# Autodesk Inventor assembly: korp
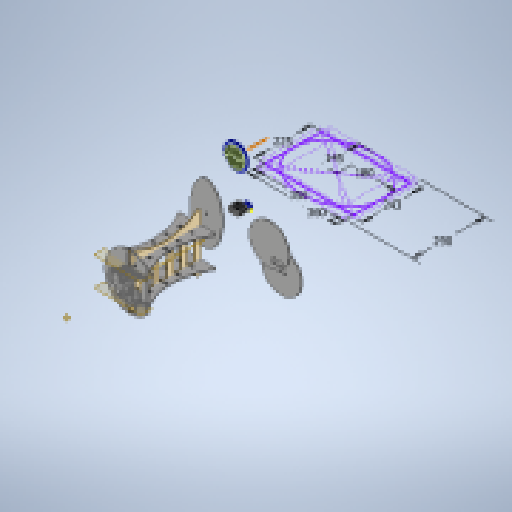
[picture p0: Inventor's stored thumbnail of the model, 512x512]
Saved by Autodesk Inventor 2023.1 (Build 271208000, 208)
## iProperties
Created: 2023-03-13
Part Number: korp
Document SubType Name: Assembly
Designer: User
Author: User
## Documents named in this file (18)
- C:\Users\DELL\reposGitHub\Cheburashka\Cheburashka_construction\korpus\korp.iam
- C:\Users\DELL\reposGitHub\Cheburashka\Cheburashka_construction\korpus\нижний эллипс тела.ipt
- C:\Users\DELL\reposGitHub\Cheburashka\Cheburashka_construction\korpus\грань тела.ipt
- C:\Users\DELL\reposGitHub\Cheburashka\Cheburashka_construction\korpus\верхний эллипс туловища.ipt
- C:\Users\DELL\reposGitHub\Cheburashka\Cheburashka_construction\korpus\нижний эллипс головы.ipt
- C:\Users\DELL\reposGitHub\Cheburashka\Cheburashka_construction\korpus\Servo.ipt
- C:\Users\DELL\reposGitHub\Cheburashka\Cheburashka_construction\korpus\Pitsco Education-739028.ipt
- C:\Users\DELL\reposGitHub\Cheburashka\Cheburashka_construction\korpus\Pitsco Education-739085.ipt
- C:\Users\DELL\reposGitHub\Cheburashka\Cheburashka_construction\korpus\трубка.ipt
- C:\Users\DELL\reposGitHub\Cheburashka\Cheburashka_construction\korpus\Prostavka.ipt
- C:\Users\DELL\reposGitHub\Cheburashka\Cheburashka_construction\korpus\лицо1.ipt
- C:\Users\DELL\reposGitHub\Cheburashka\Cheburashka_construction\korpus\att_pin.ipt
- C:\Users\DELL\reposGitHub\Cheburashka\Cheburashka_construction\platform\print\Деталь1.ipt
- C:\Users\DELL\reposGitHub\Cheburashka\Cheburashka_construction\platform\KRAVT_holder_2 (1).ipt
- C:\Users\DELL\reposGitHub\Cheburashka\Cheburashka_construction\korpus\ребро.ipt
- C:\Users\DELL\reposGitHub\Cheburashka\Cheburashka_construction\korpus\ребро_MIR.ipt
- C:\Users\DELL\reposGitHub\Cheburashka\Cheburashka_construction\korpus\креп.ipt
- C:\Users\DELL\reposGitHub\Cheburashka\Cheburashka_construction\korpus\креп_MIR.ipt
## Components (32 placed, 17 different names)
1. нижний эллипс тела:1 — Совмещение:100, Симметрия:1
2. верхний эллипс туловища:1
3. грань тела:1 — Совмещение:101, Заподлицо:19
4. нижний эллипс головы:1 — Совмещение:73
5. Pitsco Education-739028:1 — Совмещение:99
6. Pitsco Education-739085:1 — Совмещение:68, Совмещение:75, Совмещение:80
7. трубка:1 — Совмещение:68, Совмещение:74, Совмещение:81
8. Servo:4 — Совмещение:97, Совмещение:98
9. Prostavka:1 — Совмещение:73, Совмещение:74, Совмещение:75
10. Prostavka:2 — Совмещение:80, Совмещение:81, Заподлицо:16
11. лицо1:1 — Заподлицо:16, Заподлицо:17
12. att_pin:1 — Совмещение:97, Совмещение:98, Совмещение:99
13. Деталь1:1 — Заподлицо:17
14. KRAVT_holder_2 (1):1 — Совмещение:100, Совмещение:101, Симметрия:1
15. ребро:1 — Заподлицо:18, Совмещение:103, Совмещение:104, Совмещение:105, Совмещение:106, Совмещение:107, Совмещение:108, Совмещение:109, Совмещение:110, Совмещение:111, Совмещение:112, Совмещение:113, Совмещение:114, Совмещение:115, Совмещение:116, Совмещение:117, Совмещение:118
16. ребро_MIR:1 — Совмещение:102
17. креп:1 — Совмещение:105, Совмещение:106
18. креп:2 — Совмещение:103, Совмещение:104
19. креп:3 — Совмещение:107, Совмещение:108
20. креп:4 — Совмещение:109, Совмещение:110
21. креп:5 — Совмещение:111, Совмещение:112
22. креп:6 — Совмещение:113, Совмещение:114
23. креп:7 — Совмещение:117, Совмещение:118
24. креп:8 — Совмещение:115, Совмещение:116
25. креп_MIR:1
26. креп_MIR:2
27. креп_MIR:3
28. креп_MIR:4
29. креп_MIR:5
30. креп_MIR:6
31. креп_MIR:7
32. креп_MIR:8
## Relationships (33: Mate 28, Flush 4, Symmetry 1)
- Совмещение:68 [Mate]: Pitsco Education-739085:1 ↔ трубка:1
- Совмещение:73 [Mate]: нижний эллипс головы:1 ↔ Prostavka:1
- Совмещение:74 [Mate]: трубка:1 ↔ Prostavka:1
- Совмещение:75 [Mate]: Pitsco Education-739085:1 ↔ Prostavka:1
- Совмещение:80 [Mate]: Pitsco Education-739085:1 ↔ Prostavka:2
- Совмещение:81 [Mate]: трубка:1 ↔ Prostavka:2
- Заподлицо:16 [Flush]: Prostavka:2 ↔ лицо1:1
- Совмещение:97 [Mate]: Servo:4 ↔ att_pin:1
- Совмещение:98 [Mate]: Servo:4 ↔ att_pin:1
- Совмещение:99 [Mate]: Pitsco Education-739028:1 ↔ att_pin:1
- Заподлицо:17 [Flush]: лицо1:1 ↔ Деталь1:1
- Совмещение:100 [Mate]: нижний эллипс тела:1 ↔ KRAVT_holder_2 (1):1
- Совмещение:101 [Mate] (56.5 mm): грань тела:1 ↔ KRAVT_holder_2 (1):1
- Симметрия:1 [Symmetry]: нижний эллипс тела:1 ↔ KRAVT_holder_2 (1):1
- Заподлицо:18 [Flush]: ребро:1
- Заподлицо:19 [Flush] (-22.5399 mm): грань тела:1
- Совмещение:102 [Mate]: ребро_MIR:1
- Совмещение:103 [Mate]: ребро:1 ↔ креп:2
- Совмещение:104 [Mate]: ребро:1 ↔ креп:2
- Совмещение:105 [Mate]: ребро:1 ↔ креп:1
- Совмещение:106 [Mate]: ребро:1 ↔ креп:1
- Совмещение:107 [Mate]: ребро:1 ↔ креп:3
- Совмещение:108 [Mate]: ребро:1 ↔ креп:3
- Совмещение:109 [Mate]: ребро:1 ↔ креп:4
- Совмещение:110 [Mate]: ребро:1 ↔ креп:4
- Совмещение:111 [Mate]: ребро:1 ↔ креп:5
- Совмещение:112 [Mate]: ребро:1 ↔ креп:5
- Совмещение:113 [Mate]: ребро:1 ↔ креп:6
- Совмещение:114 [Mate]: ребро:1 ↔ креп:6
- Совмещение:115 [Mate]: ребро:1 ↔ креп:8
- Совмещение:116 [Mate]: ребро:1 ↔ креп:8
- Совмещение:117 [Mate]: ребро:1 ↔ креп:7
- Совмещение:118 [Mate]: ребро:1 ↔ креп:7
